# Autodesk Inventor assembly: switch
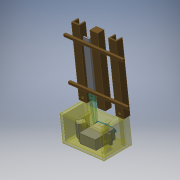
[picture p0: Inventor's stored thumbnail of the model, 180x180]
Saved by Autodesk Inventor 2018 (Build 220112000, 112)
## iProperties
Created: 2017-12-10
Part Number: switch
Document SubType Name: Assembly
Designer: ragna
Author: ragna
## Documents named in this file (9)
- C:\dev\git\tufftuff\switch.iam
- C:\dev\git\tufftuff\servo.ipt
- C:\dev\git\tufftuff\stick.ipt
- C:\dev\git\tufftuff\tracks.ipt
- C:\dev\git\tufftuff\switcher.ipt
- C:\dev\git\tufftuff\jack.ipt
- C:\dev\git\tufftuff\poker.ipt
- C:\dev\git\tufftuff\pin.ipt
- C:\dev\git\tufftuff\switchcase.ipt
## Components (8 placed, 8 different names)
1. servo:1 — Rotational:1, Mate:1
2. stick:1 — Rotational:1, Cylindrical:2, Mate:3
3. tracks:1 — Slider:1, Mate:1, Mate:4
4. switcher:1 — Slider:1, Tangent:1, Tangent:2, Mate:2
5. jack:1 — Cylindrical:3
6. poker:1 — Cylindrical:1, Tangent:1, Tangent:2, Mate:2, Mate:3
7. pin:1 — Cylindrical:1, Cylindrical:2
8. switchcase:1 — Mate:4, Cylindrical:3
## Relationships (11: Mate 4, CylindricalJoint 3, Tangent 2, RevoluteJoint 1, TranslationJoint 1)
- Rotational:1 [RevoluteJoint]: servo:1 ↔ stick:1
- Slider:1 [TranslationJoint] (0.5 mm): tracks:1 ↔ switcher:1
- Mate:1: servo:1 ↔ tracks:1
- Cylindrical:1: poker:1 ↔ pin:1
- Cylindrical:2: stick:1 ↔ pin:1
- Tangent:1: switcher:1 ↔ poker:1
- Tangent:2: switcher:1 ↔ poker:1
- Mate:2: switcher:1 ↔ poker:1
- Mate:3: stick:1 ↔ poker:1
- Mate:4: tracks:1 ↔ switchcase:1
- Cylindrical:3: jack:1 ↔ switchcase:1
